# Autodesk Inventor assembly: Lower Goal
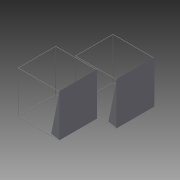
[picture p0: Inventor's stored thumbnail of the model, 180x180]
Saved by Autodesk Inventor 2014 (Build 180170000, 170)
## iProperties
Created: 2014-01-29
Part Number: Lower Goal
Document SubType Name: Assembly
Designer: NilesStanton
Author: NilesStanton
## Documents named in this file (7)
- C:\GitHub\team3566-2014\CAD\Court\Lower Goal.iam
- C:\GitHub\team3566-2014\CAD\Court\Lower Goal Longer.ipt
- C:\GitHub\team3566-2014\CAD\Court\Part4.ipt
- H:\Part1.ipt
- C:\GitHub\team3566-2014\CAD\Court\Part3.ipt
- H:\Ramp.ipt
- C:\GitHub\team3566-2014\CAD\Court\Ramp base.ipt
## Components (28 placed, 6 different names)
1. Lower Goal Longer:1 — Flush:1, Flush:2, Flush:3, Flush:4, Flush:5, Flush:6, Mate:12
2. Lower Goal Longer:2 — Flush:7, Flush:8, Flush:9
3. Part4:1 — Flush:4, Flush:5, Flush:6, Mate:3, Mate:4
4. Part4:2 — Flush:1, Flush:2, Flush:3, Flush:7, Flush:8, Flush:9
5. Lower Goal Longer:3 — Mate:6, Mate:9, Mate:13
6. Lower Goal Longer:4 — Mate:2, Mate:11
7. Part4:3 — Mate:1, Mate:5, Mate:7
8. Part4:4 — Mate:8, Mate:10
9. Part1:1
10. Part3:1 — Mate:5, Mate:6, Mate:7, Mate:14
11. Part3:2 — Mate:1, Mate:2, Mate:3, Mate:4
12. Part3:3 — Mate:10, Mate:11
13. Part3:4 — Mate:8, Mate:9
14. Ramp:1
15. Ramp base:1 — Mate:12, Mate:13, Mate:14
16. Lower Goal Longer:5
17. Lower Goal Longer:6
18. Part4:5
19. Part4:6
20. Lower Goal Longer:7
21. Lower Goal Longer:8
22. Part4:7
23. Part4:8
24. Part3:5
25. Part3:6
26. Part3:7
27. Part3:8
28. Ramp base:2
## Relationships (64: Flush 36, Mate 28)
- Flush:1: Lower Goal Longer:1 ↔ Part4:2
- Flush:2: Lower Goal Longer:1 ↔ Part4:2
- Flush:3: Lower Goal Longer:1 ↔ Part4:2
- Flush:4: Lower Goal Longer:1 ↔ Part4:1
- Flush:5: Lower Goal Longer:1 ↔ Part4:1
- Flush:6: Lower Goal Longer:1 ↔ Part4:1
- Flush:7: Lower Goal Longer:2 ↔ Part4:2
- Flush:8: Lower Goal Longer:2 ↔ Part4:2
- Flush:9: Lower Goal Longer:2 ↔ Part4:2
- [Flush]: Lower Goal Longer:3 ↔ Part4:4
- [Flush]: Lower Goal Longer:3 ↔ Part4:4
- [Flush]: Lower Goal Longer:3 ↔ Part4:4
- [Flush]: Lower Goal Longer:3 ↔ Part4:3
- [Flush]: Lower Goal Longer:3 ↔ Part4:3
- [Flush]: Lower Goal Longer:3 ↔ Part4:3
- [Flush]: Lower Goal Longer:4 ↔ Part4:4
- [Flush]: Lower Goal Longer:4 ↔ Part4:4
- [Flush]: Lower Goal Longer:4 ↔ Part4:4
- Mate:1: Part4:3 ↔ Part3:2
- Mate:2: Lower Goal Longer:4 ↔ Part3:2
- Mate:3: Part4:1 ↔ Part3:2
- Mate:4: Part4:1 ↔ Part3:2
- Mate:5: Part4:3 ↔ Part3:1
- Mate:6: Lower Goal Longer:3 ↔ Part3:1
- Mate:7: Part4:3 ↔ Part3:1
- Mate:8: Part4:4 ↔ Part3:4
- Mate:9: Lower Goal Longer:3 ↔ Part3:4
- Mate:10: Part4:4 ↔ Part3:3
- Mate:11: Lower Goal Longer:4 ↔ Part3:3
- Mate:12: Lower Goal Longer:1 ↔ Ramp base:1
- Mate:13: Lower Goal Longer:3 ↔ Ramp base:1
- Mate:14: Part3:1 ↔ Ramp base:1
- [Flush]: Lower Goal Longer:5 ↔ Part4:6
- [Flush]: Lower Goal Longer:5 ↔ Part4:6
- [Flush]: Lower Goal Longer:5 ↔ Part4:6
- [Flush]: Lower Goal Longer:5 ↔ Part4:5
- [Flush]: Lower Goal Longer:5 ↔ Part4:5
- [Flush]: Lower Goal Longer:5 ↔ Part4:5
- [Flush]: Lower Goal Longer:6 ↔ Part4:6
- [Flush]: Lower Goal Longer:6 ↔ Part4:6
- [Flush]: Lower Goal Longer:6 ↔ Part4:6
- [Flush]: Lower Goal Longer:7 ↔ Part4:8
- [Flush]: Lower Goal Longer:7 ↔ Part4:8
- [Flush]: Lower Goal Longer:7 ↔ Part4:8
- [Flush]: Lower Goal Longer:7 ↔ Part4:7
- [Flush]: Lower Goal Longer:7 ↔ Part4:7
- [Flush]: Lower Goal Longer:7 ↔ Part4:7
- [Flush]: Lower Goal Longer:8 ↔ Part4:8
- [Flush]: Lower Goal Longer:8 ↔ Part4:8
- [Flush]: Lower Goal Longer:8 ↔ Part4:8
- [Mate]: Part4:7 ↔ Part3:6
- [Mate]: Lower Goal Longer:8 ↔ Part3:6
- [Mate]: Part4:5 ↔ Part3:6
- [Mate]: Part4:5 ↔ Part3:6
- [Mate]: Part4:7 ↔ Part3:5
- [Mate]: Lower Goal Longer:7 ↔ Part3:5
- [Mate]: Part4:7 ↔ Part3:5
- [Mate]: Part4:8 ↔ Part3:8
- [Mate]: Lower Goal Longer:7 ↔ Part3:8
- [Mate]: Part4:8 ↔ Part3:7
- [Mate]: Lower Goal Longer:8 ↔ Part3:7
- [Mate]: Lower Goal Longer:5 ↔ Ramp base:2
- [Mate]: Lower Goal Longer:7 ↔ Ramp base:2
- [Mate]: Part3:5 ↔ Ramp base:2
## Named parameters: d30_d26 = 0 mm, d31_d27 = 0 mm, d32_d28 = 0 mm, d33_d29 = 0 mm, d34_d21 = 0 mm, d35_d22 = 0 mm, d36_d23 = 0 mm, d37_d24 = 0 mm, d38_d25 = 0 mm, d54_d21 = 0 mm, d55_d22 = 0 mm, d56_d23 = 0 mm, d57_d24 = 0 mm, d58_d25 = 0 mm, d59_d26 = 0 mm, d60_d27 = 0 mm, d61_d28 = 0 mm, d62_d29 = 0 mm, d63_d30_d26 = 0 mm, d64_d31_d27 = 0 mm, d65_d32_d28 = 0 mm, d66_d33_d29 = 0 mm, d67_d34_d21 = 0 mm, d68_d35_d22 = 0 mm, d69_d36_d23 = 0 mm, d70_d37_d24 = 0 mm, d71_d38_d25 = 0 mm, d72_d40 = 0 mm, d73_d41 = 0 mm, d74_d42 = 0 mm, d75_d43 = 0 mm, d76_d44 = 0 mm, d77_d45 = 0 mm, d78_d46 = 0 mm, d79_d47 = 0 mm, d80_d48 = 0 mm, d81_d49 = 0 mm, d82_d50 = 0 mm, d83_d51 = 0 mm, d84_d52 = 0 mm, d85_d53 = 0 mm
